# Autodesk Inventor assembly: motor_connect
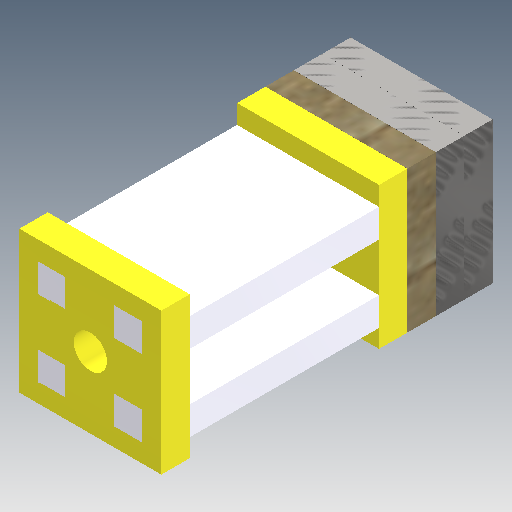
[picture p0: Inventor's stored thumbnail of the model, 512x512]
Saved by Autodesk Inventor 2020 (Build 240168000, 168)
## iProperties
Created: 2021-05-10
Part Number: motor_connect
Document SubType Name: Assembly
Designer: Hsu Daniel
Author: Hsu Daniel
## Documents named in this file (5)
- D:\Daniel\NTU\makeNTU2021\大改\motor_connect.iam
- D:\Daniel\NTU\makeNTU2021\大改\motor_bottom.ipt
- D:\Daniel\NTU\makeNTU2021\大改\motor_middle.ipt
- D:\Daniel\NTU\makeNTU2021\大改\motor_stick.ipt
- D:\Daniel\NTU\makeNTU2021\大改\motor_top.ipt
## Components (7 placed, 4 different names)
1. motor_bottom:1 — Flush:1, Flush:2, Mate:1, Flush:3, Flush:4, Flush:5, Mate:6, Mate:7, Flush:6, Flush:7, Flush:8, Flush:9, Flush:10
2. motor_bottom:2 — Flush:1, Flush:2, Mate:1, Mate:2
3. motor_middle:1 — Flush:3, Flush:4, Mate:2, Mate:8
4. motor_stick:1 — Mate:6, Flush:6, Mate:9, Mate:11
5. motor_stick:2 — Flush:5, Mate:7, Mate:10
6. motor_top:1 — Flush:9, Flush:10, Mate:11
7. motor_top:2 — Flush:7, Flush:8, Mate:8, Mate:9, Mate:10
## Relationships (18: Flush 10, Mate 8)
- Flush:1: motor_bottom:1 ↔ motor_bottom:2
- Flush:2: motor_bottom:1 ↔ motor_bottom:2
- Mate:1: motor_bottom:1 ↔ motor_bottom:2
- Flush:3: motor_bottom:1 ↔ motor_middle:1
- Flush:4: motor_bottom:1 ↔ motor_middle:1
- Mate:2: motor_bottom:2 ↔ motor_middle:1
- Flush:5: motor_bottom:1 ↔ motor_stick:2
- Mate:6: motor_bottom:1 ↔ motor_stick:1
- Mate:7: motor_bottom:1 ↔ motor_stick:2
- Flush:6: motor_bottom:1 ↔ motor_stick:1
- Flush:7: motor_bottom:1 ↔ motor_top:2
- Flush:8: motor_bottom:1 ↔ motor_top:2
- Mate:8: motor_middle:1 ↔ motor_top:2
- Flush:9: motor_bottom:1 ↔ motor_top:1
- Flush:10: motor_bottom:1 ↔ motor_top:1
- Mate:9: motor_stick:1 ↔ motor_top:2
- Mate:10: motor_stick:2 ↔ motor_top:2
- Mate:11: motor_stick:1 ↔ motor_top:1
